# Autodesk Inventor assembly: UpperJawAssembly
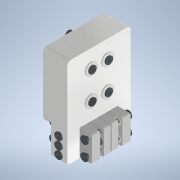
[picture p0: Inventor's stored thumbnail of the model, 180x180]
Saved by Autodesk Inventor 2022 (Build 260153000, 153)
## iProperties
Created: 2021-11-09
Part Number: UpperJawAssembly
Document SubType Name: Assembly
Designer: JK
Author: JK
## Documents named in this file (9)
- C:\Users\JK\Documents\Inventor\UTM\UpperJawAssembly.iam
- C:\Users\JK\Documents\Inventor\UTM\UpperJawSupport.ipt
- C:\Users\JK\Documents\Inventor\UTM\M5Nut.ipt
- C:\Users\JK\Documents\Inventor\UTM\M5x15BoltFlatHead.ipt
- C:\Users\JK\Documents\Inventor\UTM\UpperJaw.ipt
- C:\Users\JK\Documents\Inventor\UTM\M5 Washer.ipt
- C:\Users\JK\Documents\Inventor\UTM\PernoM5x30Plano.ipt
- C:\Users\JK\Documents\Inventor\UTM\ViseAAssembly.iam
- C:\Users\JK\Documents\Inventor\UTM\ViseBAssembly.iam
## Components (26 placed, 8 different names)
1. UpperJawSupport:1 — Coincidencia:6, Ángulo:5, Coincidencia:7, Coincidencia:8, Coincidencia:9, Coincidencia:10, Coincidencia:11, Coincidencia:12, Coincidencia:13, Coincidencia:14, Coincidencia:15
2. M5Nut:1
3. M5Nut:2
4. M5Nut:3
5. M5Nut:4
6. M5x15BoltFlatHead:1 — Coincidencia:8, Coincidencia:9, Nivelación:4
7. M5x15BoltFlatHead:2 — Coincidencia:12, Nivelación:4, Nivelación:5, Nivelación:6
8. M5x15BoltFlatHead:3 — Coincidencia:11, Nivelación:5
9. M5x15BoltFlatHead:4 — Coincidencia:10, Nivelación:6
10. UpperJaw:1 — Coincidencia:13, Coincidencia:14, Coincidencia:15, Coincidencia:16, Coincidencia:17, Coincidencia:54, Coincidencia:55, Coincidencia:56
11. ViseAAssembly:1 [sub-assembly] — Coincidencia:57
12. ViseAAssembly:2 [sub-assembly] — Coincidencia:54, Coincidencia:55, Coincidencia:56, Coincidencia:58, Coincidencia:59, Coincidencia:60
13. ViseBAssembly:1 [sub-assembly] — Coincidencia:57
14. ViseBAssembly:2 [sub-assembly] — Coincidencia:58, Coincidencia:59, Coincidencia:60
15. M5Nut:5 — Coincidencia:6, Ángulo:5, Coincidencia:7
16. M5Nut:6
17. M5Nut:7
18. M5Nut:8
19. PernoM5x30Plano:1 — Coincidencia:18, Coincidencia:19
20. M5 Washer:3 — Coincidencia:16, Coincidencia:17, Coincidencia:18, Coincidencia:19
21. PernoM5x30Plano:2
22. M5 Washer:4
23. PernoM5x30Plano:3
24. M5 Washer:5
25. PernoM5x30Plano:4
26. M5 Washer:6
## Component patterns: (4 elements, first: M5Nut:5), (4 elements, first: PernoM5x30Plano:1 + M5 Washer:3)
## Relationships (43: Mate 32, Flush 6, Angle 5)
- [Mate]: UpperJawSupport:1 ↔ M5Nut:2
- [Mate]: UpperJawSupport:1 ↔ M5Nut:1
- [Mate]: UpperJawSupport:1 ↔ M5Nut:3
- [Mate]: UpperJawSupport:1 ↔ M5Nut:4
- [Flush]: M5Nut:1 ↔ M5Nut:3
- [Flush]: M5Nut:2 ↔ M5Nut:3
- [Flush]: M5Nut:3 ↔ M5Nut:4
- [Angle] (0 deg): UpperJawSupport:1 ↔ M5Nut:3
- [Angle] (0 deg): UpperJawSupport:1 ↔ M5Nut:1
- [Angle] (0 deg): UpperJawSupport:1 ↔ M5Nut:4
- [Angle] (0 deg): UpperJawSupport:1 ↔ M5Nut:2
- [Mate]: UpperJawSupport:1 ↔ M5Nut:2
- Coincidencia:6 [Mate]: UpperJawSupport:1 ↔ M5Nut:5
- Ángulo:5 [Angle] (0 deg): UpperJawSupport:1 ↔ M5Nut:5
- Coincidencia:7 [Mate]: UpperJawSupport:1 ↔ M5Nut:5
- Coincidencia:8 [Mate]: UpperJawSupport:1 ↔ M5x15BoltFlatHead:1
- Coincidencia:9 [Mate] (6 mm): UpperJawSupport:1 ↔ M5x15BoltFlatHead:1
- Coincidencia:10 [Mate]: UpperJawSupport:1 ↔ M5x15BoltFlatHead:4
- Coincidencia:11 [Mate]: UpperJawSupport:1 ↔ M5x15BoltFlatHead:3
- Coincidencia:12 [Mate]: UpperJawSupport:1 ↔ M5x15BoltFlatHead:2
- Nivelación:4 [Flush]: M5x15BoltFlatHead:1 ↔ M5x15BoltFlatHead:2
- Nivelación:5 [Flush]: M5x15BoltFlatHead:2 ↔ M5x15BoltFlatHead:3
- Nivelación:6 [Flush]: M5x15BoltFlatHead:2 ↔ M5x15BoltFlatHead:4
- Coincidencia:13 [Mate]: UpperJawSupport:1 ↔ UpperJaw:1
- Coincidencia:14 [Mate]: UpperJawSupport:1 ↔ UpperJaw:1
- Coincidencia:15 [Mate]: UpperJawSupport:1 ↔ UpperJaw:1
- Coincidencia:16 [Mate]: UpperJaw:1 ↔ M5 Washer:3
- Coincidencia:17 [Mate]: UpperJaw:1 ↔ M5 Washer:3
- Coincidencia:18 [Mate]: PernoM5x30Plano:1 ↔ M5 Washer:3
- Coincidencia:19 [Mate]: PernoM5x30Plano:1 ↔ M5 Washer:3
- [Mate]: UpperJaw:1 ↔ ViseAAssembly:1
- [Mate]: UpperJaw:1 ↔ ViseAAssembly:1
- [Mate]: UpperJaw:1 ↔ ViseAAssembly:1
- [Mate]: UpperJaw:1 ↔ ViseAAssembly:1
- [Mate]: ViseAAssembly:1 ↔ ViseBAssembly:1
- [Mate]: ViseAAssembly:1 ↔ ViseBAssembly:1
- Coincidencia:54 [Mate]: UpperJaw:1 ↔ ViseAAssembly:2
- Coincidencia:55 [Mate]: UpperJaw:1 ↔ ViseAAssembly:2
- Coincidencia:56 [Mate]: UpperJaw:1 ↔ ViseAAssembly:2
- Coincidencia:57 [Mate]: ViseAAssembly:1 ↔ ViseBAssembly:1
- Coincidencia:58 [Mate]: ViseAAssembly:2 ↔ ViseBAssembly:2
- Coincidencia:59 [Mate]: ViseAAssembly:2 ↔ ViseBAssembly:2
- Coincidencia:60 [Mate]: ViseAAssembly:2 ↔ ViseBAssembly:2
